# Autodesk Inventor assembly: E1_Base_Meca_IIm_Ligne
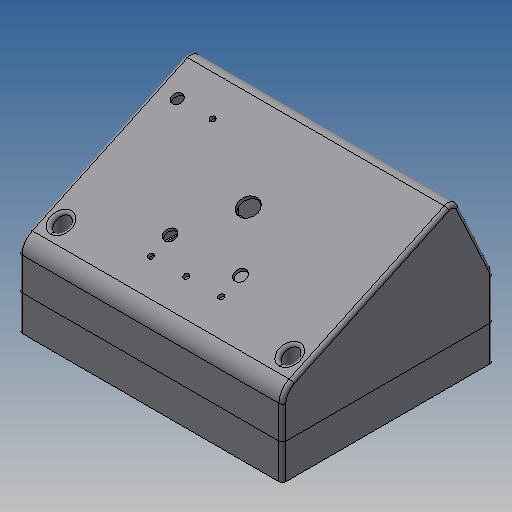
[picture p0: Inventor's stored thumbnail of the model, 512x512]
Saved by Autodesk Inventor 2025.3 (Build 293356000, 356)
## iProperties
Created: 2026-08-27
Part Number: E1_Base_Meca_IIm_Ligne
Project: Nom Projet
Description: Ens. Nom Ensemble
Document SubType Name: Assembly
Designer: jules
Mass: 6.15944 g
Surface Area: 1807.99 cm^2
Volume: 175.338 cm^3
Density: 0.035129 g/cm^3
Author: jules
## Documents named in this file (9)
- C:\Users\jules\OneDrive\PCB_Perso\PCB_IIm_Ligne\Meca_IIm_Ligne\E1_Base_Meca_IIm_Ligne.iam
- C:\Users\jules\OneDrive\PCB_Perso\PCB_IIm_Ligne\Meca_IIm_Ligne\Base_Meca_IIm_Ligne.ipt
- C:\Users\jules\OneDrive\PCB_Perso\PCB_IIm_Ligne\Meca_IIm_Ligne\Leste_Meca_IIm_Ligne.ipt
- C:\Users\jules\OneDrive\PCB_Perso\PCB_IIm_Ligne\Meca_IIm_Ligne\StandardParts\Visserie\ISO4032_Ecrou\ISO4032_M3.ipt
- C:\Users\jules\OneDrive\PCB_Perso\PCB_IIm_Ligne\Meca_IIm_Ligne\StandardParts\Visserie\ISO4032_Ecrou.ipt
- C:\Users\jules\OneDrive\PCB_Perso\PCB_IIm_Ligne\Meca_IIm_Ligne\StandardParts\Visserie\ISO4762\ISO4762_M3x5.ipt
- C:\Users\jules\OneDrive\PCB_Perso\PCB_IIm_Ligne\Meca_IIm_Ligne\StandardParts\Visserie\ISO4762.ipt
- C:\Users\jules\OneDrive\PCB_Perso\PCB_IIm_Ligne\Meca_IIm_Ligne\StandardParts\Visserie\ISO4762\ISO4762_M3x10.ipt
- C:\Users\jules\OneDrive\PCB_Perso\PCB_IIm_Ligne\Meca_IIm_Ligne\Couvercle_Meca_IIm_Ligne.ipt
## Components (15 placed, 6 different names)
1. Base_Meca_IIm_Ligne:1 — Placage:1, Placage:2, Placage:3, Placage:4, Placage:5, Placage:6, Placage:11, Placage:12, Placage:13, Placage:14, Placage:15, Placage:16, Placage:17, Placage:18, Angle:3, Placage:20, Angle:4, Placage:22, Placage:24, Placage:25, Placage:26, Placage:28, Placage:29, Placage:32, Placage:33, Placage:36, Placage:37, Placage:38
2. Leste_Meca_IIm_Ligne:1 — Placage:1, Placage:2, Placage:3, Placage:7, Placage:8, Placage:9, Placage:10, Angle:1, Angle:2
3. ISO4032_M3:1 — Placage:4, Placage:5, Placage:6
4. ISO4032_M3:2 — Placage:21, Angle:4, Placage:22
5. ISO4032_M3:3 — Placage:24, Placage:25, Placage:26
6. ISO4032_M3:4 — Placage:27, Placage:28, Placage:29
7. ISO4032_M3:5 — Placage:19, Angle:3, Placage:20
8. ISO4032_M3:6 — Placage:31, Placage:32, Placage:33
9. ISO4762_M3x5:4 — Placage:9, Placage:10, Angle:1, Placage:21
10. ISO4762_M3x5:5 — Placage:7, Placage:8, Angle:2, Placage:19
11. ISO4762_M3x10:6 — Placage:15, Placage:16, Placage:27
12. ISO4762_M3x10:7 — Placage:14, Placage:17
13. ISO4762_M3x10:8 — Placage:11, Placage:12
14. ISO4762_M3x10:9 — Placage:13, Placage:18, Placage:31
15. Couvercle_Meca_IIm_Ligne:1 — Placage:36, Placage:37, Placage:38
## Relationships (38: Mate 34, Angle 4)
- Placage:1 [Mate]: Base_Meca_IIm_Ligne:1 ↔ Leste_Meca_IIm_Ligne:1
- Placage:2 [Mate]: Base_Meca_IIm_Ligne:1 ↔ Leste_Meca_IIm_Ligne:1
- Placage:3 [Mate]: Base_Meca_IIm_Ligne:1 ↔ Leste_Meca_IIm_Ligne:1
- Placage:4 [Mate]: Base_Meca_IIm_Ligne:1 ↔ ISO4032_M3:1
- Placage:5 [Mate]: Base_Meca_IIm_Ligne:1 ↔ ISO4032_M3:1
- Placage:6 [Mate]: Base_Meca_IIm_Ligne:1 ↔ ISO4032_M3:1
- Placage:7 [Mate]: Leste_Meca_IIm_Ligne:1 ↔ ISO4762_M3x5:5
- Placage:8 [Mate]: Leste_Meca_IIm_Ligne:1 ↔ ISO4762_M3x5:5
- Placage:9 [Mate]: Leste_Meca_IIm_Ligne:1 ↔ ISO4762_M3x5:4
- Placage:10 [Mate]: Leste_Meca_IIm_Ligne:1 ↔ ISO4762_M3x5:4
- Angle:1 (0 deg): Leste_Meca_IIm_Ligne:1 ↔ ISO4762_M3x5:4
- Angle:2 (0 deg): Leste_Meca_IIm_Ligne:1 ↔ ISO4762_M3x5:5
- Placage:11 [Mate]: Base_Meca_IIm_Ligne:1 ↔ ISO4762_M3x10:8
- Placage:12 [Mate] (1.6 mm): Base_Meca_IIm_Ligne:1 ↔ ISO4762_M3x10:8
- Placage:13 [Mate]: Base_Meca_IIm_Ligne:1 ↔ ISO4762_M3x10:9
- Placage:14 [Mate]: Base_Meca_IIm_Ligne:1 ↔ ISO4762_M3x10:7
- Placage:15 [Mate]: Base_Meca_IIm_Ligne:1 ↔ ISO4762_M3x10:6
- Placage:16 [Mate] (1.6 mm): Base_Meca_IIm_Ligne:1 ↔ ISO4762_M3x10:6
- Placage:17 [Mate] (1.6 mm): Base_Meca_IIm_Ligne:1 ↔ ISO4762_M3x10:7
- Placage:18 [Mate] (1.6 mm): Base_Meca_IIm_Ligne:1 ↔ ISO4762_M3x10:9
- Placage:19 [Mate]: ISO4032_M3:5 ↔ ISO4762_M3x5:5
- Angle:3 (0 deg): Base_Meca_IIm_Ligne:1 ↔ ISO4032_M3:5
- Placage:20 [Mate]: Base_Meca_IIm_Ligne:1 ↔ ISO4032_M3:5
- Placage:21 [Mate]: ISO4032_M3:2 ↔ ISO4762_M3x5:4
- Angle:4 (0 deg): Base_Meca_IIm_Ligne:1 ↔ ISO4032_M3:2
- Placage:22 [Mate]: Base_Meca_IIm_Ligne:1 ↔ ISO4032_M3:2
- Placage:24 [Mate] (1 mm): Base_Meca_IIm_Ligne:1 ↔ ISO4032_M3:3
- Placage:25 [Mate]: Base_Meca_IIm_Ligne:1 ↔ ISO4032_M3:3
- Placage:26 [Mate]: Base_Meca_IIm_Ligne:1 ↔ ISO4032_M3:3
- Placage:27 [Mate]: ISO4032_M3:4 ↔ ISO4762_M3x10:6
- Placage:28 [Mate]: Base_Meca_IIm_Ligne:1 ↔ ISO4032_M3:4
- Placage:29 [Mate]: Base_Meca_IIm_Ligne:1 ↔ ISO4032_M3:4
- Placage:31 [Mate]: ISO4032_M3:6 ↔ ISO4762_M3x10:9
- Placage:32 [Mate]: Base_Meca_IIm_Ligne:1 ↔ ISO4032_M3:6
- Placage:33 [Mate]: Base_Meca_IIm_Ligne:1 ↔ ISO4032_M3:6
- Placage:36 [Mate]: Base_Meca_IIm_Ligne:1 ↔ Couvercle_Meca_IIm_Ligne:1
- Placage:37 [Mate]: Base_Meca_IIm_Ligne:1 ↔ Couvercle_Meca_IIm_Ligne:1
- Placage:38 [Mate]: Base_Meca_IIm_Ligne:1 ↔ Couvercle_Meca_IIm_Ligne:1
